# Autodesk Inventor assembly: Cockpit_side_frame
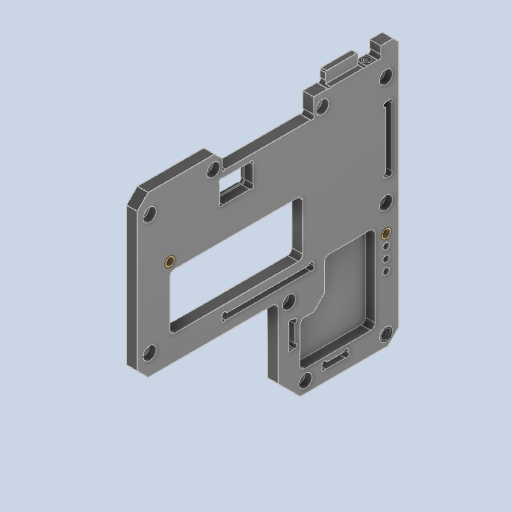
[picture p0: Inventor's stored thumbnail of the model, 512x512]
Saved by Autodesk Inventor 2022.5 (Build 265521000, 521)
## iProperties
Created: 2023-05-18
Part Number: Cockpit_side_frame
Document SubType Name: Assembly
Designer: Masato Kubotera
Author: Masato Kubotera
## Documents named in this file (6)
- C:\Users\Masato\Documents\Inventor\SUSTAINA-OP\ModelingFiles\UpperBody\Cockpit\Cockpit_side_frame.iam
- C:\Users\Masato\Documents\Inventor\SUSTAINA-OP\ModelingFiles\UpperBody\Cockpit\Cockpit_side_frame.ipt
- C:\Users\Masato\Documents\Inventor\SUSTAINA-OP\ModelingFiles\COTS\Neodymium_magnet_Phi3_T3.ipt
- C:\Users\Masato\Documents\Inventor\SUSTAINA-OP\ModelingFiles\COTS\InsertNut\UD-43040.ipt
- C:\Users\Masato\Documents\Inventor\SUSTAINA-OP\ModelingFiles\COTS\Spacer\BRU-305.ipt
- C:\Users\Masato\Documents\Inventor\SUSTAINA-OP\ModelingFiles\COTS\InsertNut\IRU-304S.ipt
## Components (8 placed, 5 different names)
1. Cockpit_side_frame:1 — Insert:1, Insert:2, Insert:3, Insert:4, Insert:5, Insert:6, Insert:7
2. Neodymium_magnet_Phi3_T3:1 — Insert:1
3. Neodymium_magnet_Phi3_T3:2 — Insert:2
4. Neodymium_magnet_Phi3_T3:3 — Insert:3
5. UD-43040:1 — Insert:4
6. BRU-305:1 — Insert:5
7. IRU-304S:1 — Insert:6
8. UD-43040:2 — Insert:7
## Relationships (7: Insert 7)
- Insert:1: Cockpit_side_frame:1 ↔ Neodymium_magnet_Phi3_T3:1
- Insert:2: Cockpit_side_frame:1 ↔ Neodymium_magnet_Phi3_T3:2
- Insert:3: Cockpit_side_frame:1 ↔ Neodymium_magnet_Phi3_T3:3
- Insert:4: Cockpit_side_frame:1 ↔ UD-43040:1
- Insert:5: Cockpit_side_frame:1 ↔ BRU-305:1
- Insert:6: Cockpit_side_frame:1 ↔ IRU-304S:1
- Insert:7: Cockpit_side_frame:1 ↔ UD-43040:2
